# Autodesk Inventor assembly: BobbinGuide
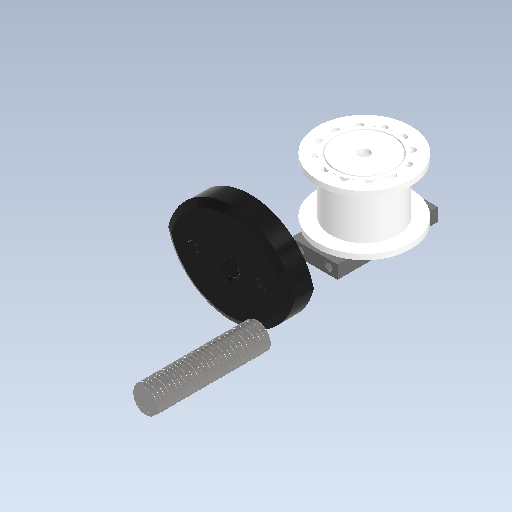
[picture p0: Inventor's stored thumbnail of the model, 512x512]
Saved by Autodesk Inventor 2021 (Build 250183000, 183)
## iProperties
Created: 2020-03-09
Part Number: BobbinGuide
Document SubType Name: Assembly
Designer: elmar
Author: elmar
## Documents named in this file (7)
- D:\FourWireBraidingMachine\InventorFiles\Carriage.iam
- D:\FourWireBraidingMachine\InventorFiles\CarriagePlate.ipt
- D:\FourWireBraidingMachine\InventorFiles\SpoolHolder.ipt
- D:\FourWireBraidingMachine\InventorFiles\Spool.ipt
- D:\FourWireBraidingMachine\InventorFiles\Spring.ipt
- D:\FourWireBraidingMachine\InventorFiles\SpoolSpringBushing.ipt
- D:\FourWireBraidingMachine\InventorFiles\M8_34mmRod.ipt
## Components (6 placed, 6 different names)
1. CarriagePlate:1 — Insert:21, Angle:1
2. SpoolHolder:1 — Insert:20, Insert:21, Angle:1
3. Spool:1 — Mate:1, Mate:5, Insert:20, Insert:22
4. Spring:1 — Mate:1, Mate:5
5. SpoolSpringBushing:1 — Insert:22
6. M8_34mmRod:1
## Relationships (6: Insert 3, Mate 2, Angle 1)
- Mate:1: Spool:1 ↔ Spring:1
- Mate:5: Spool:1 ↔ Spring:1
- Insert:20: SpoolHolder:1 ↔ Spool:1
- Insert:21: CarriagePlate:1 ↔ SpoolHolder:1
- Insert:22: Spool:1 ↔ SpoolSpringBushing:1
- Angle:1 (0 deg): CarriagePlate:1 ↔ SpoolHolder:1
